# Autodesk Inventor assembly: SMALLER
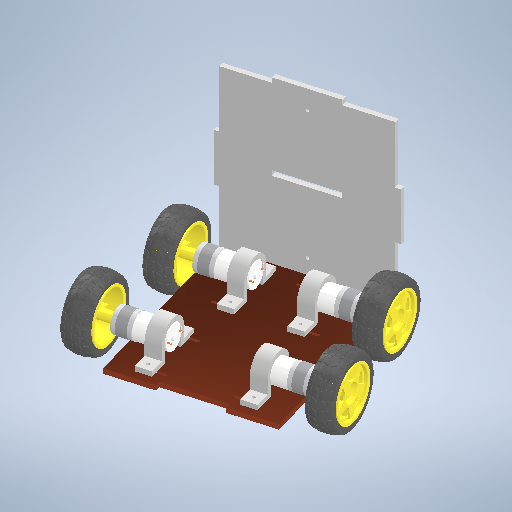
[picture p0: Inventor's stored thumbnail of the model, 512x512]
Saved by Autodesk Inventor 2025.3 (Build 293356030, 356C)
## iProperties
Created: 2026-06-30
Part Number: SMALLER
Document SubType Name: Assembly
Designer: user
Author: user
## Documents named in this file (4)
- C:\Docs\shcool\dojo\Design_3\Smaller\SMALLER.iam
- C:\Docs\shcool\dojo\Design_3\Smaller\WHEEL_BASE.iam
- C:\Docs\shcool\dojo\Design_3\Smaller\back.ipt
- C:\Docs\shcool\dojo\Design_3\Smaller\Fastener.ipt
## Components (3 placed, 3 different names)
1. WHEEL_BASE:1 [sub-assembly] — Mate:3, Mate:4
2. back:1 — Mate:1, Mate:2
3. Fastener:1 — Mate:1, Mate:2, Mate:3, Mate:4
## Relationships (4: Mate 4)
- Mate:1: back:1 ↔ Fastener:1
- Mate:2: back:1 ↔ Fastener:1
- Mate:3: WHEEL_BASE:1 ↔ Fastener:1
- Mate:4: WHEEL_BASE:1 ↔ Fastener:1
